# Autodesk Inventor assembly: 全体
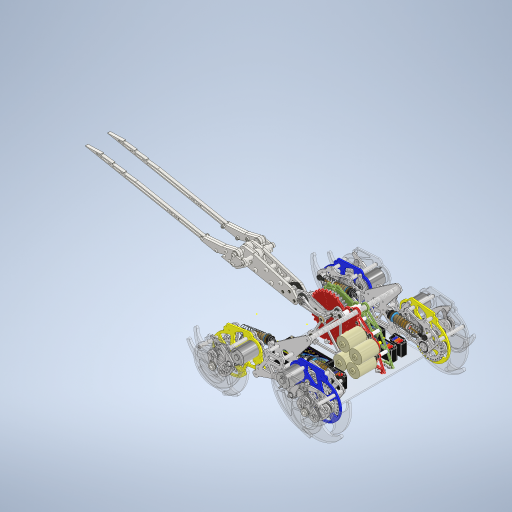
[picture p0: Inventor's stored thumbnail of the model, 512x512]
Saved by Autodesk Inventor 2023 (Build 270158000, 158)
## iProperties
Created: 2022-05-13
Part Number: 全体
Document SubType Name: Assembly
Designer: muzho
Author: muzho
## Documents named in this file (8)
- C:\Users\muzho\Documents\srdc\srdc_2\全体.iam
- C:\Users\muzho\Documents\srdc\srdc_2\脚\足全体.iam
- C:\Users\muzho\Documents\srdc\srdc_reference\院2年機 中型ミドルロッド(2020 9 20更新)\アーム アームユニットアセンブリ.iam
- C:\Users\muzho\Documents\srdc\srdc_2\バッテリー BAKUSO.ipt
- C:\Users\muzho\Documents\srdc\srdc_2\MC402CR.ipt
- C:\Users\muzho\Documents\srdc\srdc_2\脚\足全体_temp.iam
- C:\Users\muzho\Documents\srdc\srdc_2\脚\シャフト.ipt
- C:\Users\muzho\Documents\srdc\srdc_2\下板.ipt
## Components (10 placed, 7 different names)
1. 足全体:2 [sub-assembly] — メイト:1, メイト:2, メイト:3, 挿入:2, フラッシュ:7
2. アーム アームユニットアセンブリ:1 [sub-assembly] — フラッシュ:6, メイト:5, メイト:6, 角度:1, フラッシュ:7
3. バッテリー BAKUSO:1 — フラッシュ:4, メイト:4
4. バッテリー BAKUSO:2 — メイト:7
5. MC402CR:1 — メイト:8
6. MC402CR:2 — メイト:9
7. MC402CR:3 — フラッシュ:4, メイト:10
8. 足全体_temp:1 [sub-assembly] — メイト:1, メイト:2, メイト:3, 挿入:1, フラッシュ:5, 挿入:2
9. シャフト:1 — 挿入:1, メイト:5, メイト:6
10. 下板:1 — フラッシュ:5, フラッシュ:6, メイト:4, 角度:1, メイト:7, メイト:8, メイト:9, メイト:10
## Relationships (17: Mate 10, Flush 4, Insert 2, Angle 1)
- フラッシュ:4 [Flush]: バッテリー BAKUSO:1 ↔ MC402CR:3
- メイト:1 [Mate] (-320 mm): 足全体:2 ↔ 足全体_temp:1
- メイト:2 [Mate]: 足全体:2 ↔ 足全体_temp:1
- メイト:3 [Mate]: 足全体:2 ↔ 足全体_temp:1
- 挿入:1 [Insert]: 足全体_temp:1 ↔ シャフト:1
- フラッシュ:5 [Flush]: 足全体_temp:1 ↔ 下板:1
- フラッシュ:6 [Flush]: アーム アームユニットアセンブリ:1 ↔ 下板:1
- 挿入:2 [Insert]: 足全体:2 ↔ 足全体_temp:1
- メイト:4 [Mate]: バッテリー BAKUSO:1 ↔ 下板:1
- メイト:5 [Mate]: アーム アームユニットアセンブリ:1 ↔ シャフト:1
- メイト:6 [Mate]: アーム アームユニットアセンブリ:1 ↔ シャフト:1
- 角度:1 [Angle] (180 deg): アーム アームユニットアセンブリ:1 ↔ 下板:1
- フラッシュ:7 [Flush] (-70 mm): 足全体:2 ↔ アーム アームユニットアセンブリ:1
- メイト:7 [Mate]: バッテリー BAKUSO:2 ↔ 下板:1
- メイト:8 [Mate]: MC402CR:1 ↔ 下板:1
- メイト:9 [Mate]: MC402CR:2 ↔ 下板:1
- メイト:10 [Mate]: MC402CR:3 ↔ 下板:1
